# Autodesk Inventor assembly: Assembly1
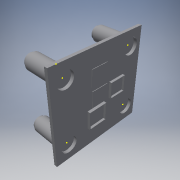
[picture p0: Inventor's stored thumbnail of the model, 180x180]
Saved by Autodesk Inventor 2019 (Build 230136000, 136)
## iProperties
Created: 2020-02-19
Part Number: Assembly1
Document SubType Name: Assembly
Designer: Goutam Joshi
Author: Goutam Joshi
## Documents named in this file (4)
- E:\Assembly1.iam
- E:\cofee table.ipt
- E:\blocks.ipt
- E:\table leg.ipt
## Components (14 placed, 3 different names)
1. cofee table:1 — Rotational:1, Rigid:1, Rotational:2, Rigid:2, Rigid:3, Mate:1
2. blocks:1
3. blocks:2 — Flush:1
4. blocks:3 — Mate:1, Flush:1
5. blocks:4
6. blocks:5
7. blocks:6
8. blocks:7
9. blocks:8 — Rigid:3
10. table leg:1 — Rotational:1
11. table leg:2 — Rigid:1
12. table leg:3 — Rotational:2
13. table leg:4 — Rigid:2
14. blocks:9
## Relationships (7: WeldJoint 3, RevoluteJoint 2, Mate 1, Flush 1)
- Rotational:1 [RevoluteJoint]: cofee table:1 ↔ table leg:1
- Rigid:1 [WeldJoint]: cofee table:1 ↔ table leg:2
- Rotational:2 [RevoluteJoint]: cofee table:1 ↔ table leg:3
- Rigid:2 [WeldJoint]: cofee table:1 ↔ table leg:4
- Rigid:3 [WeldJoint]: cofee table:1 ↔ blocks:8
- Mate:1: cofee table:1 ↔ blocks:3
- Flush:1: blocks:2 ↔ blocks:3
